# Autodesk Inventor assembly: Piasta_koła_tylnego
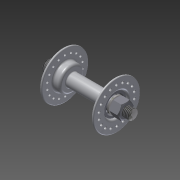
[picture p0: Inventor's stored thumbnail of the model, 180x180]
Saved by Autodesk Inventor 2015 (Build 190159000, 159)
## iProperties
Created: 2015-11-24
Part Number: Piasta_koła_tylnego
Document SubType Name: Assembly
Designer: graaapsik
Author: graaapsik
## Documents named in this file (8)
- C:\Users\EriveltonDell\Documents\Centro Universitário da FEI\Wheelchair\CADEIRA DE RODAS - DESENHO\Model\Piasta_koła_tylnego.iam
- Piasta.iam
- C:\Users\EriveltonDell\Documents\Centro Universitário da FEI\Wheelchair\CADEIRA DE RODAS - DESENHO\Model\Korpus_piasty_koła_tylnego.ipt
- C:\Users\EriveltonDell\Documents\Centro Universitário da FEI\Wheelchair\CADEIRA DE RODAS - DESENHO\Model\Oś_piasty_koła_tylnego.ipt
- C:\Users\EriveltonDell\Documents\Centro Universitário da FEI\Wheelchair\CADEIRA DE RODAS - DESENHO\Model\ISO 4034 - M12ISO.ipt
- C:\Users\EriveltonDell\Documents\Centro Universitário da FEI\Wheelchair\CADEIRA DE RODAS - DESENHO\Model\ISO 7092 - ST 12 - 140 HV.ipt
- C:\Users\EriveltonDell\Documents\Centro Universitário da FEI\Wheelchair\CADEIRA DE RODAS - DESENHO\Model\Rolling bearing QJ1001 GB_T 294-94.ipt
- C:\Users\EriveltonDell\Documents\Centro Universitário da FEI\Wheelchair\CADEIRA DE RODAS - DESENHO\Model\ISO 4145 Tuleja redukcyjna N4 3_8 x 1_4.ipt
## Components (8 placed, 6 different names)
1. Oś_piasty_koła_tylnego:1 — Walcowe:1
2. Korpus_piasty_koła_tylnego:1 — Walcowe:1, Wstaw:1, Wstaw:4
3. Rolling bearing GB/T 294-1994 QJ1001:3 — Wstaw:1, Wstaw:2
4. Rolling bearing GB/T 294-1994 QJ1001:4 — Wstaw:4, Wstaw:5
5. ISO 7092 ST 12 - 140 HV:3 — Wstaw:2, Wstaw:6
6. ISO 7092 ST 12 - 140 HV:4 — Wstaw:5, Wstaw:7
7. ISO 4034 M12:2 — Wstaw:6
8. ISO 4145 Tuleja redukcyjna N4 3/8 x 1/4:2 — Wstaw:7
## Relationships (7: Insert 6, CylindricalJoint 1)
- Walcowe:1 [CylindricalJoint]: Oś_piasty_koła_tylnego:1 ↔ Korpus_piasty_koła_tylnego:1
- Wstaw:1 [Insert]: Korpus_piasty_koła_tylnego:1 ↔ Rolling bearing GB/T 294-1994 QJ1001:3
- Wstaw:2 [Insert]: Rolling bearing GB/T 294-1994 QJ1001:3 ↔ ISO 7092 ST 12 - 140 HV:3
- Wstaw:4 [Insert]: Korpus_piasty_koła_tylnego:1 ↔ Rolling bearing GB/T 294-1994 QJ1001:4
- Wstaw:5 [Insert]: Rolling bearing GB/T 294-1994 QJ1001:4 ↔ ISO 7092 ST 12 - 140 HV:4
- Wstaw:6 [Insert]: ISO 7092 ST 12 - 140 HV:3 ↔ ISO 4034 M12:2
- Wstaw:7 [Insert]: ISO 7092 ST 12 - 140 HV:4 ↔ ISO 4145 Tuleja redukcyjna N4 3/8 x 1/4:2
